# Autodesk Inventor assembly: ThighLeftNCS
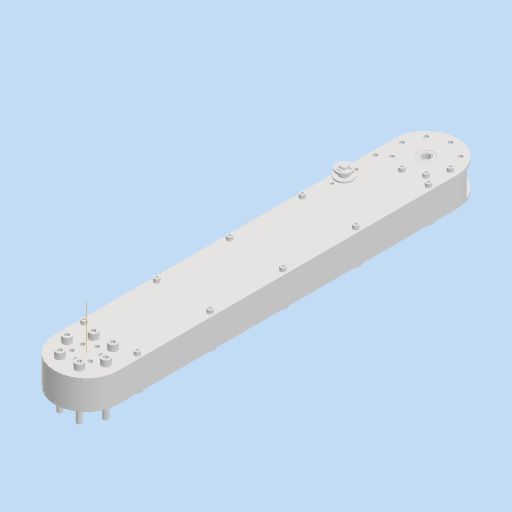
[picture p0: Inventor's stored thumbnail of the model, 512x512]
Saved by Autodesk Inventor 2023 (Build 270158000, 158)
## iProperties
Created: 2026-06-18
Part Number: ThighLeftNCS
Document SubType Name: Assembly
Designer: Nathann
Author: Nathann
## Documents named in this file (2)
- C:\Users\Nathann\ClawdDrive\Objet3D\RunningRobot\PartURDF\ThighLeftNCS.iam
- C:\Users\Nathann\ClawdDrive\Objet3D\RunningRobot\PartURDF\ThighLeft.iam
## Components (1 placed, 1 different names)
1. ThighLeft:1 [sub-assembly] — Mate:1, Mate:2, Angle:1
## Relationships (5: Mate 4, Angle 1)
- Mate:1: ThighLeft:1
- Mate:2: ThighLeft:1
- Mate:3
- Mate:4
- Angle:1 (180 deg): ThighLeft:1
